# Autodesk Inventor assembly: Harmonic Mount Box Assembly
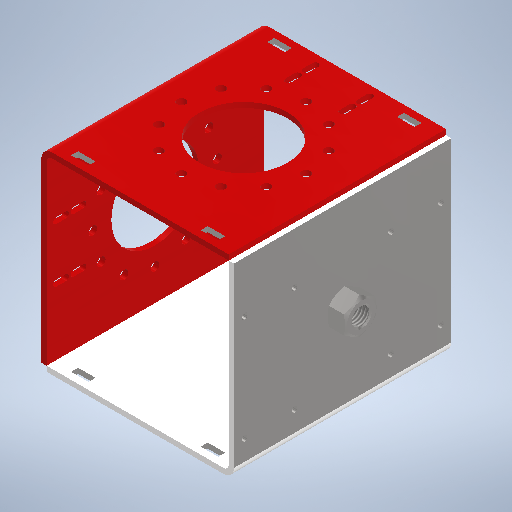
[picture p0: Inventor's stored thumbnail of the model, 512x512]
Saved by Autodesk Inventor 2025 (Build 290162000, 162)
## iProperties
Created: 2025-08-10
Part Number: Harmonic Mount Box Assembly
Document SubType Name: Assembly
Designer: yshis
Author: yshis
## Documents named in this file (4)
- C:\Users\yshis\Documents\Harmonic Drive Mount\Harmonic Mount Box Assembly.iam
- C:\Users\yshis\Documents\Harmonic Drive Mount\Face with Harmonic Drive.ipt
- C:\Users\yshis\Documents\Harmonic Drive Mount\Face with CWT hole.ipt
- C:\Users\yshis\Documents\Inventor\Content Center Files\R2025\en-US\DIN EN ISO 4032\DIN EN ISO 4032 - M12.ipt
## Components (3 placed, 3 different names)
1. Face with Harmonic Drive:1 — Mate:1, Mate:2, Flush:1
2. Face with CWT hole:1 — Mate:1, Mate:2, Flush:1, Mate:3, Mate:4, Mate:5
3. DIN EN ISO 4032 M12:1 — Mate:3, Mate:4, Mate:5
## Relationships (6: Mate 5, Flush 1)
- Mate:1: Face with Harmonic Drive:1 ↔ Face with CWT hole:1
- Mate:2: Face with Harmonic Drive:1 ↔ Face with CWT hole:1
- Flush:1: Face with Harmonic Drive:1 ↔ Face with CWT hole:1
- Mate:3: Face with CWT hole:1 ↔ DIN EN ISO 4032 M12:1
- Mate:4 (-55 mm): Face with CWT hole:1 ↔ DIN EN ISO 4032 M12:1
- Mate:5 (-62 mm): Face with CWT hole:1 ↔ DIN EN ISO 4032 M12:1
